# Autodesk Inventor assembly: Montagem
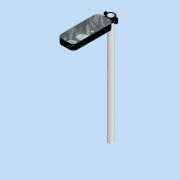
[picture p0: Inventor's stored thumbnail of the model, 180x180]
Saved by Autodesk Inventor 2022 (Build 260153000, 153)
## iProperties
Created: 2022-09-16
Part Number: Montagem
Document SubType Name: Assembly
Designer: aleal
Author: aleal
## Documents named in this file (11)
- C:\Users\aleal\Desktop\Wellison EC\Montagem.iam
- C:\Users\aleal\Desktop\Wellison EC\Part1.ipt
- C:\Users\aleal\Desktop\Wellison EC\Part2.ipt
- C:\Users\aleal\Desktop\Wellison EC\Part3.ipt
- C:\Users\aleal\Desktop\Wellison EC\Part4.ipt
- C:\Users\aleal\Desktop\Wellison EC\Part5.ipt
- C:\Users\aleal\Desktop\Wellison EC\Part6.ipt
- C:\Users\aleal\Documents\Inventor\Content Center Files\R2022\en-US\BS EN ISO 4762\BS EN ISO 4762 - M5 x 25(1).ipt
- C:\Users\aleal\Documents\Inventor\Content Center Files\R2022\en-US\CNS 3129\CNS 3129 - M 5 x 0,8.ipt
- C:\Users\aleal\Documents\Inventor\Content Center Files\R2022\en-US\CNS 3130\CNS 3130 - M 5.ipt
- C:\Users\aleal\Documents\Inventor\Content Center Files\R2022\en-US\BS 4183(5)\BS 4183 - M3 x 10(2) I.ipt
## Components (18 placed, 10 different names)
1. Part1:1 — Flush:1, Flush:2, Mate:1, Mate:15, Mate:16, Flush:8, Flush:9, Flush:10, Flush:11
2. Part2:1 — Flush:1, Flush:2, Mate:1, Mate:2, Flush:3, Flush:4, Mate:11, Mate:14, Mate:17
3. Part3:1 — Mate:2, Flush:3, Flush:4, Mate:4, Flush:7, Mate:6, Mate:7, Mate:8, Mate:9
4. Part5:1 — Mate:4, Flush:7
5. BS EN ISO 4762 - Metric M5 x 25:1 — Mate:6, Mate:7, Mate:12, Mate:13
6. BS EN ISO 4762 - Metric M5 x 25:2 — Mate:8, Mate:9, Mate:10
7. CNS 3129 M 5:1 — Mate:10, Mate:11
8. CNS 3130 M 5:1 — Mate:12, Mate:13, Mate:14
9. BS 4183 Slotted Cheese Head Machine Screw - Metric M3 x 10:1
10. BS 4183 Slotted Cheese Head Machine Screw - Metric M3 x 10:2
11. BS 4183 Slotted Cheese Head Machine Screw - Metric M3 x 10:3
12. BS 4183 Slotted Cheese Head Machine Screw - Metric M3 x 10:6
13. BS 4183 Slotted Cheese Head Machine Screw - Metric M3 x 10:7
14. BS 4183 Slotted Cheese Head Machine Screw - Metric M3 x 10:8
15. BS 4183 Slotted Cheese Head Machine Screw - Metric M3 x 10:11
16. BS 4183 Slotted Cheese Head Machine Screw - Metric M3 x 10:12
17. Part4:1 — Mate:15, Mate:16, Flush:8, Flush:9
18. Part6:1 — Mate:17, Flush:10, Flush:11
## Relationships (24: Mate 15, Flush 9)
- Flush:1: Part1:1 ↔ Part2:1
- Flush:2: Part1:1 ↔ Part2:1
- Mate:1: Part1:1 ↔ Part2:1
- Mate:2: Part2:1 ↔ Part3:1
- Flush:3: Part2:1 ↔ Part3:1
- Flush:4: Part2:1 ↔ Part3:1
- Mate:4: Part3:1 ↔ Part5:1
- Flush:7: Part3:1 ↔ Part5:1
- Mate:6: Part3:1 ↔ BS EN ISO 4762 - Metric M5 x 25:1
- Mate:7: Part3:1 ↔ BS EN ISO 4762 - Metric M5 x 25:1
- Mate:8: Part3:1 ↔ BS EN ISO 4762 - Metric M5 x 25:2
- Mate:9: Part3:1 ↔ BS EN ISO 4762 - Metric M5 x 25:2
- Mate:10: BS EN ISO 4762 - Metric M5 x 25:2 ↔ CNS 3129 M 5:1
- Mate:11: Part2:1 ↔ CNS 3129 M 5:1
- Mate:12: BS EN ISO 4762 - Metric M5 x 25:1 ↔ CNS 3130 M 5:1
- Mate:13: BS EN ISO 4762 - Metric M5 x 25:1 ↔ CNS 3130 M 5:1
- Mate:14: Part2:1 ↔ CNS 3130 M 5:1
- Mate:15: Part1:1 ↔ Part4:1
- Mate:16: Part1:1 ↔ Part4:1
- Flush:8: Part1:1 ↔ Part4:1
- Flush:9: Part1:1 ↔ Part4:1
- Mate:17: Part2:1 ↔ Part6:1
- Flush:10: Part1:1 ↔ Part6:1
- Flush:11: Part1:1 ↔ Part6:1
